# Autodesk Inventor assembly: se300-t-b
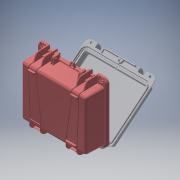
[picture p0: Inventor's stored thumbnail of the model, 180x180]
Saved by Autodesk Inventor 2019.4 (Build 234330000, 330)
## iProperties
Created: 2021-02-08
Part Number: se300-t-b
Document SubType Name: Assembly
Designer: Jorian Brusind
Sending System: SOLIDWORKS 2017-2017109
MC: AMD64
MC_MODEL: Intel64 Family 6 Model 60 Stepping 3, GenuineIntel
OS: Windows_NT
FRU: Parasolid Version 29.0, build 195, 12- 2-2016
FORMAT: text
GUISE: transmit
KEY: 300-ASSY-Rev Q
FILE: 300-ASSY-Rev Q.x_t
DATE: Wed Aug 09 09:25:08 2017
Author: Jorian Brusind
## Documents named in this file (4)
- C:\Users\Jorian Brusind\Documents\GitHub\PersonalProjects\HyperRail\Inventor Files\se300-t-b.iam
- C:\Users\Jorian Brusind\Documents\GitHub\PersonalProjects\HyperRail\Inventor Files\7310_300_Bottom_Rev-M_4-7-17(Default).ipt
- C:\Users\Jorian Brusind\Documents\GitHub\PersonalProjects\HyperRail\Inventor Files\7310_300_Bottom_Rev-M_4-7-17(Default)_1.ipt
- C:\Users\Jorian Brusind\Documents\GitHub\PersonalProjects\HyperRail\Inventor Files\7300 300_Top_Rev M(Default).ipt
## Components (3 placed, 3 different names)
1. 7310_300_Bottom_Rev-M_4-7-17(Default)
2. 7310_300_Bottom_Rev-M_4-7-17(Default)_1 — Mate:1, Mate:2
3. 7300 300_Top_Rev M(Default) — Mate:1, Mate:2
## Relationships (2: Mate 2)
- Mate:1: 7310_300_Bottom_Rev-M_4-7-17(Default)_1 ↔ 7300 300_Top_Rev M(Default)
- Mate:2: 7310_300_Bottom_Rev-M_4-7-17(Default)_1 ↔ 7300 300_Top_Rev M(Default)
